# Autodesk Inventor assembly: Robotic Arm 3D Model
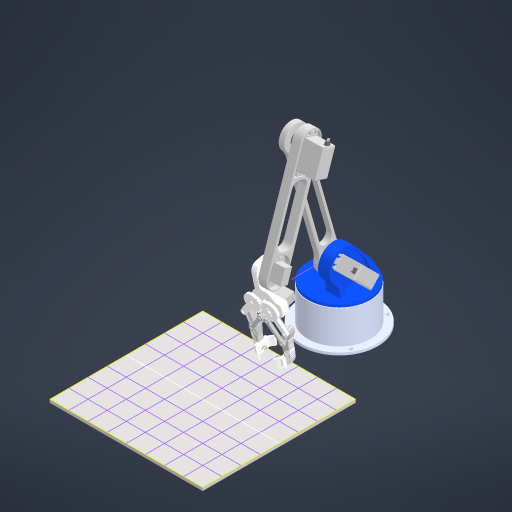
[picture p0: Inventor's stored thumbnail of the model, 512x512]
Saved by Autodesk Inventor 2024 (Build 280153000, 153)
## iProperties
Company: Unknown organisation
Created: 2023-03-04
Part Number: Robotic Arm 3D Model
Description: HOOPS Exchange Step
Document SubType Name: Assembly
Designer: hrush
Authority: Unknown authorisation
Sending System: HOOPS Exchange
Preprocessor: HOOPS Exchange 2022.1
Title: /tmp/filefZVxeh/Robotic Arm 3D Model.step
Author: root
## Documents named in this file (9)
- P:\Arduino\chessbot\data\cad\inventor\Charm Assembly.iam
- P:\Arduino\chessbot\data\cad\inventor\Gripper Assembly.iam
- P:\Arduino\chessbot\data\cad\inventor\Servo Motor Micro  9g.ipt
- P:\Arduino\chessbot\data\cad\inventor\Servo Motor MG996R.ipt
- P:\Arduino\chessbot\data\cad\inventor\Waist.ipt
- P:\Arduino\chessbot\data\cad\inventor\Base.ipt
- P:\Arduino\chessbot\data\cad\inventor\Arm 01-large.ipt
- P:\Arduino\chessbot\data\cad\inventor\Arm 02-large.ipt
- P:\Arduino\chessbot\data\cad\inventor\chessboard.ipt
## Components (10 placed, 10 different names)
1. Gripper Assembly_1 [sub-assembly] — Rotational:3
2. Servo Motor MG996R_13 — Mate:10, Mate:11, Mate:12, Rotational:2
3. Waist_17 — Mate:4, Mate:5, Mate:7, Mate:8, Mate:9
4. Servo Motor Micro  9g_18 — Mate:13, Mate:14, Mate:15, Rotational:3
5. Base_19 — Mate:1, Mate:2, Mate:3, Mate:16, Mate:17
6. Servo Motor MG996R_20 — Mate:7, Mate:8, Mate:9, Rotational:1
7. Servo Motor MG996R_21 — Mate:1, Mate:2, Mate:3, Mate:4, Mate:5
8. Arm 01-large:1 — Rotational:1, Rotational:2
9. Arm 02-large:1 — Mate:10, Mate:11, Mate:12, Mate:13, Mate:14, Mate:15
10. chessboard:1 — Angle:1, Mate:18, Mate:19
## Relationships (22: Mate 18, RevoluteJoint 3, Angle 1)
- Mate:1: Base_19 ↔ Servo Motor MG996R_21
- Mate:2: Base_19 ↔ Servo Motor MG996R_21
- Mate:3: Base_19 ↔ Servo Motor MG996R_21
- Mate:4: Waist_17 ↔ Servo Motor MG996R_21
- Mate:5: Waist_17 ↔ Servo Motor MG996R_21
- Mate:7: Waist_17 ↔ Servo Motor MG996R_20
- Mate:8: Waist_17 ↔ Servo Motor MG996R_20
- Mate:9: Waist_17 ↔ Servo Motor MG996R_20
- Rotational:1 [RevoluteJoint]: Servo Motor MG996R_20 ↔ Arm 01-large:1
- Mate:10: Servo Motor MG996R_13 ↔ Arm 02-large:1
- Mate:11: Servo Motor MG996R_13 ↔ Arm 02-large:1
- Mate:12: Servo Motor MG996R_13 ↔ Arm 02-large:1
- Rotational:2 [RevoluteJoint]: Servo Motor MG996R_13 ↔ Arm 01-large:1
- Mate:13: Servo Motor Micro  9g_18 ↔ Arm 02-large:1
- Mate:14: Servo Motor Micro  9g_18 ↔ Arm 02-large:1
- Mate:15: Servo Motor Micro  9g_18 ↔ Arm 02-large:1
- Rotational:3 [RevoluteJoint]: Gripper Assembly_1 ↔ Servo Motor Micro  9g_18
- Mate:16: Base_19
- Mate:17: Base_19
- Angle:1 (0 deg): chessboard:1
- Mate:18: chessboard:1
- Mate:19: chessboard:1
